# Autodesk Inventor assembly: 3D_PCB4_2024-01-15
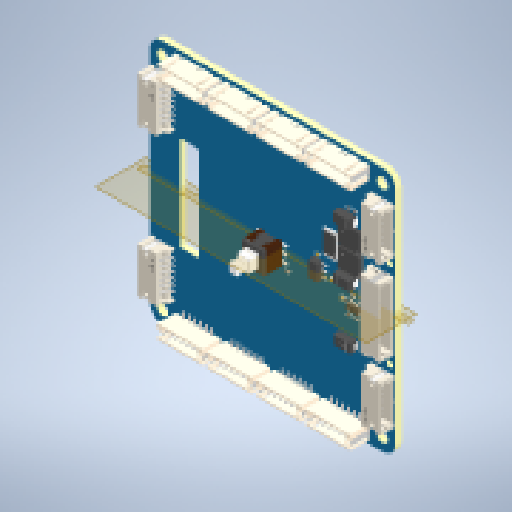
[picture p0: Inventor's stored thumbnail of the model, 512x512]
Saved by Autodesk Inventor 2024.2 (Build 282272000, 272)
## iProperties
Created: 2025-09-19
Part Number: 3D_PCB4_2024-01-15
Document SubType Name: Assembly
Designer: AdminForWorker
Title: 3D_PCB4_2024-01-15 v3
Author: AdminForWorker
## Documents named in this file (36)
- D:\dog\fox\construction\fox\boards\3D_PCB4_2024-01-15 v3.iam
- D:\dog\fox\construction\fox\boards\Board.ipt
- D:\dog\fox\construction\fox\boards\Q2.iam
- D:\dog\fox\construction\fox\boards\Q1.iam
- D:\dog\fox\construction\fox\boards\SW1.iam
- D:\dog\fox\construction\fox\boards\R15.iam
- D:\dog\fox\construction\fox\boards\U40.iam
- D:\dog\fox\construction\fox\boards\U42.iam
- D:\dog\fox\construction\fox\boards\D3.iam
- D:\dog\fox\construction\fox\boards\D2.iam
- D:\dog\fox\construction\fox\boards\R16.iam
- D:\dog\fox\construction\fox\boards\R12.iam
- D:\dog\fox\construction\fox\boards\R8.iam
- D:\dog\fox\construction\fox\boards\R9.iam
- D:\dog\fox\construction\fox\boards\R11.iam
- D:\dog\fox\construction\fox\boards\R14.iam
- D:\dog\fox\construction\fox\boards\R17.iam
- D:\dog\fox\construction\fox\boards\R22.iam
- D:\dog\fox\construction\fox\boards\R7.iam
- D:\dog\fox\construction\fox\boards\CN17.iam
- D:\dog\fox\construction\fox\boards\CN7.iam
- D:\dog\fox\construction\fox\boards\CN9.iam
- D:\dog\fox\construction\fox\boards\CN10.iam
- D:\dog\fox\construction\fox\boards\CN12.iam
- D:\dog\fox\construction\fox\boards\CN13.iam
- D:\dog\fox\construction\fox\boards\CN15.iam
- D:\dog\fox\construction\fox\boards\CN16.iam
- D:\dog\fox\construction\fox\boards\CN6.iam
- D:\dog\fox\construction\fox\boards\C50.iam
- D:\dog\fox\construction\fox\boards\C52.iam
- D:\dog\fox\construction\fox\boards\C51.iam
- D:\dog\fox\construction\fox\boards\D4.iam
- D:\dog\fox\construction\fox\boards\CN8.iam
- D:\dog\fox\construction\fox\boards\CN11.iam
- D:\dog\fox\construction\fox\boards\CN14.iam
- D:\dog\fox\construction\fox\boards\CN5.iam
## Components (35 placed, 35 different names)
1. Board:1 — Угол:1
2. Q2:1 [sub-assembly]
3. Q1:1 [sub-assembly]
4. SW1:1 [sub-assembly] — Совмещение:1
5. R15:1 [sub-assembly]
6. U40:1 [sub-assembly]
7. U42:1 [sub-assembly]
8. D3:1 [sub-assembly]
9. D2:1 [sub-assembly]
10. R16:1 [sub-assembly]
11. R12:1 [sub-assembly]
12. R8:1 [sub-assembly]
13. R9:1 [sub-assembly]
14. R11:1 [sub-assembly]
15. R14:1 [sub-assembly]
16. R17:1 [sub-assembly]
17. R22:1 [sub-assembly]
18. R7:1 [sub-assembly]
19. CN17:1 [sub-assembly]
20. CN7:1 [sub-assembly]
21. CN9:1 [sub-assembly]
22. CN10:1 [sub-assembly]
23. CN12:1 [sub-assembly]
24. CN13:1 [sub-assembly]
25. CN15:1 [sub-assembly]
26. CN16:1 [sub-assembly]
27. CN6:1 [sub-assembly]
28. C50:1 [sub-assembly]
29. C52:1 [sub-assembly]
30. C51:1 [sub-assembly]
31. D4:1 [sub-assembly]
32. CN8:1 [sub-assembly]
33. CN11:1 [sub-assembly]
34. CN14:1 [sub-assembly]
35. CN5:1 [sub-assembly]
## Relationships (2: Mate 1, Angle 1)
- Совмещение:1 [Mate]: SW1:1
- Угол:1 [Angle] (0 deg): Board:1
